# Autodesk Inventor assembly: MotorAssemblyV3
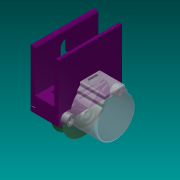
[picture p0: Inventor's stored thumbnail of the model, 180x180]
Saved by Autodesk Inventor 2013 (Build 170138000, 138)
## iProperties
Created: 2013-08-17
Part Number: MotorAssemblyV3
Document SubType Name: Assembly
Designer: Sawaiz
Author: Sawaiz
## Documents named in this file (5)
- S:\Sawaiz\Documents\3D Modeling\Inventor\PolarGraph\MotorAssemblyV3.iam
- S:\Sawaiz\Documents\3D Modeling\Inventor\PolarGraph\MotorClipV3.iam
- S:\Sawaiz\Documents\3D Modeling\Inventor\PolarGraph\MotorFilamentSpool.iam
- S:\Sawaiz\Documents\3D Modeling\Inventor\Content Center Files\R2013\en-US\ANSI B18.3(05)\ANSI B18.3 - 8-32 UNC - 0.75(31).ipt
- S:\Sawaiz\Documents\3D Modeling\Inventor\PolarGraph\Imported Components\91841A009\91841A009.ipt
## Components (6 placed, 4 different names)
1. MotorClipV3:1 [sub-assembly] — Mate:1, Mate:2, Mate:3, Mate:4, Mate:5, Mate:6, Mate:7, Mate:8, Mate:9, Mate:11, Mate:12
2. MotorFilamentSpool:1 [sub-assembly] — Mate:1, Mate:2, Mate:3, Mate:10, Flush:1
3. Hexagon Socket Head Cap Screw - Inch No. 8 - 32 UNC - 3/4:1 — Mate:9, Mate:10
4. Hexagon Socket Head Cap Screw - Inch No. 8 - 32 UNC - 3/4:2 — Mate:8, Flush:1
5. 91841A009:1 — Mate:5, Mate:7, Mate:11
6. 91841A009:2 — Mate:4, Mate:6, Mate:12
## Relationships (13: Mate 12, Flush 1)
- Mate:1: MotorClipV3:1 ↔ MotorFilamentSpool:1
- Mate:2: MotorClipV3:1 ↔ MotorFilamentSpool:1
- Mate:3: MotorClipV3:1 ↔ MotorFilamentSpool:1
- Mate:4: MotorClipV3:1 ↔ 91841A009:2
- Mate:5: MotorClipV3:1 ↔ 91841A009:1
- Mate:6: MotorClipV3:1 ↔ 91841A009:2
- Mate:7: MotorClipV3:1 ↔ 91841A009:1
- Mate:8: MotorClipV3:1 ↔ Hexagon Socket Head Cap Screw - Inch No. 8 - 32 UNC - 3/4:2
- Mate:9: MotorClipV3:1 ↔ Hexagon Socket Head Cap Screw - Inch No. 8 - 32 UNC - 3/4:1
- Mate:10: MotorFilamentSpool:1 ↔ Hexagon Socket Head Cap Screw - Inch No. 8 - 32 UNC - 3/4:1
- Flush:1: MotorFilamentSpool:1 ↔ Hexagon Socket Head Cap Screw - Inch No. 8 - 32 UNC - 3/4:2
- Mate:11: MotorClipV3:1 ↔ 91841A009:1
- Mate:12: MotorClipV3:1 ↔ 91841A009:2
